# Autodesk Inventor assembly: finalized collector and pan
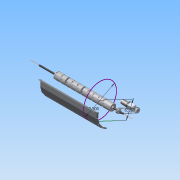
[picture p0: Inventor's stored thumbnail of the model, 180x180]
Saved by Autodesk Inventor 2015 (Build 190159000, 159)
## iProperties
Created: 2017-01-28
Part Number: finalized collector and pan
Document SubType Name: Assembly
Designer: nick pc
Author: nick pc
## Documents named in this file (7)
- D:\robotics\finalized collector and pan.iam
- D:\robotics\plate.ipt
- D:\robotics\BRUCES ROLLER.ipt
- D:\robotics\Imported Components\.5 HEX BEARING\.5 HEX BEARING.ipt
- D:\robotics\Imported Components\thunder hex\thunder hex.ipt
- D:\robotics\belts and pullys.iam
- D:\robotics\Imported Components\v2-VersaPlanetary-1stage-with-AM9015-20131031\v2-VersaPlanetary-1stage-with-AM9015-20131031.iam
## Components (7 placed, 6 different names)
1. plate:1 — Rotational:1, Rotational:2
2. BRUCES ROLLER:1 — Rotational:1
3. .5 HEX BEARING:1 — Rotational:3
4. .5 HEX BEARING:2 — Rotational:4
5. thunder hex:1 — Rotational:2, Rotational:3, Rotational:4, Mate:1, Mate:2
6. belts and pullys:1 [sub-assembly] — Mate:1, Mate:2, Mate:3, Mate:4
7. v2-VersaPlanetary-1stage-with-AM9015-20131031:1 [sub-assembly] — Mate:3, Mate:4
## Relationships (9: RevoluteJoint 4, Mate 4, Flush 1)
- Flush:5 (94.742 mm)
- Rotational:1 [RevoluteJoint] (127 mm): plate:1 ↔ BRUCES ROLLER:1
- Rotational:2 [RevoluteJoint] (228.6 mm): plate:1 ↔ thunder hex:1
- Rotational:3 [RevoluteJoint] (101.6 mm): .5 HEX BEARING:1 ↔ thunder hex:1
- Rotational:4 [RevoluteJoint] (165.1 mm): .5 HEX BEARING:2 ↔ thunder hex:1
- Mate:1: thunder hex:1 ↔ belts and pullys:1
- Mate:2: thunder hex:1 ↔ belts and pullys:1
- Mate:3: belts and pullys:1 ↔ v2-VersaPlanetary-1stage-with-AM9015-20131031:1
- Mate:4: belts and pullys:1 ↔ v2-VersaPlanetary-1stage-with-AM9015-20131031:1
